# Autodesk Inventor assembly: Assembly5
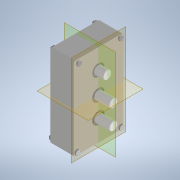
[picture p0: Inventor's stored thumbnail of the model, 180x180]
Saved by Autodesk Inventor 2021 (Build 250183000, 183)
## iProperties
Created: 2023-06-22
Part Number: Assembly5
Document SubType Name: Assembly
Designer: mahmo
Author: mahmo
## Documents named in this file (9)
- D:\AsU\gearbox\Assembly5.iam
- D:\AsU\gearbox\gears_bot.iam
- D:\AsU\gearbox\gears_up.iam
- D:\AsU\gearbox\Shaft1.ipt
- C:\Users\mahmo\OneDrive\Documents\Inventor\Content Center Files\R2021\en-US\BS 290 SKF(30)\BS 290 SKF - SKF 61805.ipt
- D:\AsU\gearbox\casing_MIR.ipt
- D:\AsU\gearbox\casing_MIR_MIR.ipt
- C:\Users\mahmo\OneDrive\Documents\Inventor\Content Center Files\R2021\en-US\BS EN 24017\ISO 4017 - M8 x 80BS EN.ipt
- C:\Users\mahmo\OneDrive\Documents\Inventor\Content Center Files\R2021\en-US\AS 1112 (2)\AS 1112 - M8  Type 8.ipt
## Components (21 placed, 8 different names)
1. gears_bot:1 [sub-assembly] — Mate:1, Mate:2, Mate:3, Mate:4
2. gears_up:1 [sub-assembly] — Mate:5, Mate:6, Mate:7, Mate:8
3. Shaft:1 — Mate:3, Mate:4, Mate:6, Mate:7, Mate:15, Mate:19
4. Shaft:2 — Mate:1, Mate:2, Mate:16, Mate:17
5. Shaft:3 — Mate:5, Mate:8, Mate:13, Mate:21
6. BS 290 SKF 61805:1 — Mate:13
7. BS 290 SKF 61805:2 — Mate:16
8. BS 290 SKF 61805:3 — Mate:15
9. casing_MIR:1 — Flush:4, Flush:5, Flush:6, Mate:18, Mate:20, Mate:22, Mate:32, Mate:34, Mate:36, Mate:38
10. BS 290 SKF 61805:4 — Mate:19, Mate:20
11. BS 290 SKF 61805:5 — Mate:21, Mate:22
12. BS 290 SKF 61805:6 — Mate:17, Mate:18
13. casing_MIR_MIR:1 — Flush:7, Flush:8, Flush:9, Mate:23, Mate:24, Mate:25, Mate:26, Mate:27, Mate:28, Mate:29, Mate:30
14. BS EN 24017 - Metric M8 x 80:1 — Mate:23, Mate:24, Mate:31
15. BS EN 24017 - Metric M8 x 80:2 — Mate:25, Mate:26, Mate:33
16. BS EN 24017 - Metric M8 x 80:3 — Mate:29, Mate:30, Mate:35
17. BS EN 24017 - Metric M8 x 80:4 — Mate:27, Mate:28, Mate:37
18. AS 1112 (2) - Metric M8  Type 8:1 — Mate:31, Mate:32
19. AS 1112 (2) - Metric M8  Type 8:2 — Mate:33, Mate:34
20. AS 1112 (2) - Metric M8  Type 8:3 — Mate:35, Mate:36
21. AS 1112 (2) - Metric M8  Type 8:4 — Mate:37, Mate:38
## Relationships (39: Mate 33, Flush 6)
- Mate:1: gears_bot:1 ↔ Shaft:2
- Mate:2: gears_bot:1 ↔ Shaft:2
- Mate:3: gears_bot:1 ↔ Shaft:1
- Mate:4: gears_bot:1 ↔ Shaft:1
- Mate:5: gears_up:1 ↔ Shaft:3
- Mate:6: gears_up:1 ↔ Shaft:1
- Mate:7 (5 mm): gears_up:1 ↔ Shaft:1
- Mate:8: gears_up:1 ↔ Shaft:3
- Mate:13: Shaft:3 ↔ BS 290 SKF 61805:1
- Mate:15: Shaft:1 ↔ BS 290 SKF 61805:3
- Mate:16: Shaft:2 ↔ BS 290 SKF 61805:2
- Flush:4: casing_MIR:1
- Flush:5: casing_MIR:1
- Flush:6: casing_MIR:1
- Mate:17: Shaft:2 ↔ BS 290 SKF 61805:6
- Mate:18: casing_MIR:1 ↔ BS 290 SKF 61805:6
- Mate:19: Shaft:1 ↔ BS 290 SKF 61805:4
- Mate:20: casing_MIR:1 ↔ BS 290 SKF 61805:4
- Mate:21: Shaft:3 ↔ BS 290 SKF 61805:5
- Mate:22: casing_MIR:1 ↔ BS 290 SKF 61805:5
- Flush:7: casing_MIR_MIR:1
- Flush:8: casing_MIR_MIR:1
- Flush:9: casing_MIR_MIR:1
- Mate:23: casing_MIR_MIR:1 ↔ BS EN 24017 - Metric M8 x 80:1
- Mate:24: casing_MIR_MIR:1 ↔ BS EN 24017 - Metric M8 x 80:1
- Mate:25: casing_MIR_MIR:1 ↔ BS EN 24017 - Metric M8 x 80:2
- Mate:26: casing_MIR_MIR:1 ↔ BS EN 24017 - Metric M8 x 80:2
- Mate:27: casing_MIR_MIR:1 ↔ BS EN 24017 - Metric M8 x 80:4
- Mate:28: casing_MIR_MIR:1 ↔ BS EN 24017 - Metric M8 x 80:4
- Mate:29: casing_MIR_MIR:1 ↔ BS EN 24017 - Metric M8 x 80:3
- Mate:30: casing_MIR_MIR:1 ↔ BS EN 24017 - Metric M8 x 80:3
- Mate:31: BS EN 24017 - Metric M8 x 80:1 ↔ AS 1112 (2) - Metric M8  Type 8:1
- Mate:32: casing_MIR:1 ↔ AS 1112 (2) - Metric M8  Type 8:1
- Mate:33: BS EN 24017 - Metric M8 x 80:2 ↔ AS 1112 (2) - Metric M8  Type 8:2
- Mate:34: casing_MIR:1 ↔ AS 1112 (2) - Metric M8  Type 8:2
- Mate:35: BS EN 24017 - Metric M8 x 80:3 ↔ AS 1112 (2) - Metric M8  Type 8:3
- Mate:36: casing_MIR:1 ↔ AS 1112 (2) - Metric M8  Type 8:3
- Mate:37: BS EN 24017 - Metric M8 x 80:4 ↔ AS 1112 (2) - Metric M8  Type 8:4
- Mate:38: casing_MIR:1 ↔ AS 1112 (2) - Metric M8  Type 8:4
